# Autodesk Inventor assembly: ArcadeController
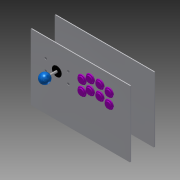
[picture p0: Inventor's stored thumbnail of the model, 180x180]
Saved by Autodesk Inventor 2013 (Build 170138000, 138)
## iProperties
Created: 2013-01-27
Part Number: ArcadeController
Document SubType Name: Assembly
Designer: xylzlyx
Author: xylzlyx
## Documents named in this file (9)
- C:\dev\pewpew\assemblies\ArcadeController.iam
- C:\dev\pewpew\parts\Panel_bottom.ipt
- C:\dev\pewpew\parts\Panel_top.ipt
- C:\dev\pewpew\parts\JLF-TP-8YT_ball.ipt
- C:\dev\pewpew\parts\JLF-TP-8YT_body.ipt
- C:\dev\pewpew\parts\JLF-TP-8YT_ring.ipt
- C:\dev\pewpew\assemblies\ArcadeController\Design Accelerator\Bolted Connection1.iam
- C:\dev\pewpew\assemblies\ArcadeController\Design Accelerator\Bolted Connection2.iam
- C:\dev\pewpew\parts\OBSF-30-B_button.ipt
## Components (15 placed, 7 different names)
1. BottomPanel:1 — Mate:1, Flush:1, Flush:2, Flush:3
2. TopPanel:1 — Flush:1, Flush:2, Flush:3, Insert:1, Mate:2, Mate:3, Mate:4, Mate:5, Insert:4, Insert:5, Insert:6, Insert:7, Insert:8, Insert:9, Insert:10, Insert:11
3. JoystickBall:1 — Insert:2
4. JLF-TP-8YT_body:1 — Insert:1, Insert:2, Insert:3
5. JoystickCover:1 — Insert:3
6. Bolted Connection:1 [sub-assembly] — Mate:2, Mate:3
7. Bolted Connection:2 [sub-assembly] — Mate:4, Mate:5
8. OBSF-30-B_button:1 — Insert:4
9. OBSF-30-B_button:2 — Insert:5
10. OBSF-30-B_button:3 — Insert:6
11. OBSF-30-B_button:4 — Insert:7
12. OBSF-30-B_button:5 — Insert:8
13. OBSF-30-B_button:6 — Insert:9
14. OBSF-30-B_button:7 — Insert:10
15. OBSF-30-B_button:8 — Insert:11
## Relationships (19: Insert 11, Mate 5, Flush 3)
- Mate:1: BottomPanel:1
- Flush:1: BottomPanel:1 ↔ TopPanel:1
- Flush:2: BottomPanel:1 ↔ TopPanel:1
- Flush:3: BottomPanel:1 ↔ TopPanel:1
- Insert:1: TopPanel:1 ↔ JLF-TP-8YT_body:1
- Insert:2: JoystickBall:1 ↔ JLF-TP-8YT_body:1
- Mate:2: TopPanel:1 ↔ Bolted Connection:1
- Mate:3: TopPanel:1 ↔ Bolted Connection:1
- Mate:4: TopPanel:1 ↔ Bolted Connection:2
- Mate:5: TopPanel:1 ↔ Bolted Connection:2
- Insert:3 (3 mm): JLF-TP-8YT_body:1 ↔ JoystickCover:1
- Insert:4: TopPanel:1 ↔ OBSF-30-B_button:1
- Insert:5: TopPanel:1 ↔ OBSF-30-B_button:2
- Insert:6: TopPanel:1 ↔ OBSF-30-B_button:3
- Insert:7: TopPanel:1 ↔ OBSF-30-B_button:4
- Insert:8: TopPanel:1 ↔ OBSF-30-B_button:5
- Insert:9: TopPanel:1 ↔ OBSF-30-B_button:6
- Insert:10: TopPanel:1 ↔ OBSF-30-B_button:7
- Insert:11: TopPanel:1 ↔ OBSF-30-B_button:8
